# Autodesk Inventor assembly: mascon
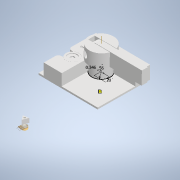
[picture p0: Inventor's stored thumbnail of the model, 180x180]
Saved by Autodesk Inventor 2021 (Build 250183000, 183)
## iProperties
Created: 2021-03-06
Part Number: mascon
Document SubType Name: Assembly
Designer: ben
Author: ben
## Documents named in this file (20)
- C:\Users\teh18\OneDrive\BVE Controller\r68-bve-mascon\mascon.iam
- C:\Users\teh18\OneDrive\BVE Controller\r68-bve-mascon\mascon.ipt
- C:\Users\teh18\OneDrive\BVE Controller\r68-bve-mascon\handle_base.ipt
- C:\Users\teh18\OneDrive\BVE Controller\r68-bve-mascon\handle.ipt
- C:\Users\teh18\OneDrive\BVE Controller\r68-bve-mascon\Compress Spring11.ipt
- C:\Users\teh18\OneDrive\BVE Controller\r68-bve-mascon\handle piston 2.ipt
- C:\Users\teh18\OneDrive\BVE Controller\r68-bve-mascon\HandleGear.ipt
- C:\Users\teh18\OneDrive\BVE Controller\r68-bve-mascon\EncoderGear.ipt
- C:\Users\teh18\OneDrive\BVE Controller\Reverser.ipt
- C:\Users\teh18\OneDrive\BVE Controller\HandleNotchRod.ipt
- C:\Users\teh18\OneDrive\BVE Controller\ReverserGear.ipt
- C:\Users\teh18\OneDrive\BVE Controller\ReverserRack.ipt
- C:\Users\teh18\OneDrive\BVE Controller\potentiometer-b10k-1.snapshot.2\PotentiometerB10K.ipt
- C:\Users\teh18\OneDrive\BVE Controller\r68-bve-mascon\HandlePotAttachmentGear.ipt
- C:\Users\teh18\OneDrive\BVE Controller\r68-bve-mascon\mascon\AIP\FEA\djp8lvgqo.fins
- C:\Users\teh18\OneDrive\BVE Controller\r68-bve-mascon\mascon\AIP\FEA\djp8lvgww.fsat
- C:\Users\teh18\OneDrive\BVE Controller\r68-bve-mascon\mascon\AIP\FEA\djp8lvgww.ftes
- C:\Users\teh18\OneDrive\BVE Controller\r68-bve-mascon\mascon\AIP\FEA\djp8lvgxs.fwiz
- C:\Users\teh18\OneDrive\BVE Controller\r68-bve-mascon\mascon\AIP\FEA\djp8lvhwg.fmsh
- C:\Users\teh18\OneDrive\BVE Controller\r68-bve-mascon\mascon\AIP\FEA\djp8lvhwh.fres
## Components (13 placed, 13 different names)
1. mascon:1 — Mate:2, lever handle
2. handle_base:1 — Mate:2, lever handle, deadman switch, Mate:4, Mate:5, Mate:6, Flush:1, Mate:8
3. handle:1 — deadman switch, Tangent:1
4. Compress Spring1:1 — Mate:4, Mate:5
5. handle piston 2:1 — Tangent:1, Mate:6
6. HandleGear:1 — Flush:1, Mate:7
7. EncoderGear:1
8. Reverser:1 — Flush:5, Mate:9
9. HandleNotchRod:1
10. ReverserGear:1 — Flush:5, Flush:6, Tangent:2, Mate:9
11. ReverserRack:1 — Mate:7, Mate:8, Flush:6, Tangent:2
12. PotentiometerB10K:1 — Flush:7
13. HandlePotAttachmentGear:1 — Flush:7
## Relationships (15: Mate 7, Flush 4, RevoluteJoint 2, Tangent 2)
- Mate:2: mascon:1 ↔ handle_base:1
- lever handle [RevoluteJoint]: mascon:1 ↔ handle_base:1
- deadman switch [RevoluteJoint] (-1 mm): handle_base:1 ↔ handle:1
- Mate:4: handle_base:1 ↔ Compress Spring1:1
- Mate:5: handle_base:1 ↔ Compress Spring1:1
- Tangent:1: handle:1 ↔ handle piston 2:1
- Mate:6: handle_base:1 ↔ handle piston 2:1
- Flush:1: handle_base:1 ↔ HandleGear:1
- Flush:5: Reverser:1 ↔ ReverserGear:1
- Mate:7: HandleGear:1 ↔ ReverserRack:1
- Mate:8: handle_base:1 ↔ ReverserRack:1
- Flush:6: ReverserGear:1 ↔ ReverserRack:1
- Tangent:2: ReverserGear:1 ↔ ReverserRack:1
- Mate:9: Reverser:1 ↔ ReverserGear:1
- Flush:7: PotentiometerB10K:1 ↔ HandlePotAttachmentGear:1
